# Autodesk Inventor assembly: CubliAssembly2
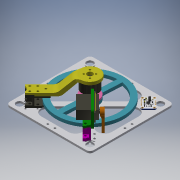
[picture p0: Inventor's stored thumbnail of the model, 180x180]
Saved by Autodesk Inventor 2018 (Build 220112000, 112)
## iProperties
Created: 2019-06-12
Part Number: CubliAssembly2
Document SubType Name: Assembly
Designer: anirudh
Author: anirudh
## Documents named in this file (13)
- C:\Users\anirudh\Documents\MARS Fund\Cubli\CAD Files\CubliAssembly2.iam
- C:\Users\anirudh\Documents\MARS Fund\Cubli\CAD Files\SidePanel.ipt
- C:\Users\anirudh\Documents\MARS Fund\Cubli\CAD Files\MountingBracket.ipt
- C:\Users\anirudh\Documents\MARS Fund\Cubli\CAD Files\MountingArm.ipt
- C:\Users\anirudh\Documents\MARS Fund\Cubli\CAD Files\SnailMotorModel.ipt
- C:\Users\anirudh\Documents\MARS Fund\Cubli\CAD Files\MotorMountingHub.ipt
- C:\Users\anirudh\Documents\MARS Fund\Cubli\CAD Files\AssaultReaper500Servo.ipt
- C:\Users\anirudh\Documents\MARS Fund\Cubli\CAD Files\ServoMount.ipt
- C:\Users\anirudh\Documents\MARS Fund\Cubli\CAD Files\ServoBase.ipt
- C:\Users\anirudh\Documents\MARS Fund\Cubli\CAD Files\Adafruit_BNO055_AP214.ipt
- C:\Users\anirudh\Documents\MARS Fund\Cubli\CAD Files\FlywheelMount.ipt
- C:\Users\anirudh\Documents\MARS Fund\Cubli\CAD Files\AcrylicFlywheels\AcrylicFlywheel3.ipt
- C:\Users\anirudh\Documents\MARS Fund\Cubli\CAD Files\Brake2.ipt
## Components (12 placed, 12 different names)
1. SidePanel:1 — Mate:3, Mate:11, Mate:12, Mate:13, Mate:21, Mate:27, Mate:28, Mate:32, Mate:33, Mate:38, Mate:39
2. MountingBracket:1 — Mate:3, Mate:6, Flush:1, Mate:34, Mate:38, Mate:39
3. MountingArm:1 — Mate:6, Flush:1, Mate:9, Mate:34, Mate:35
4. SnailMotorModel:1 — Mate:7, Mate:8, Mate:9, Mate:35
5. MotorMountingHub:1 — Mate:7, Mate:8
6. AssaultReaper500Servo:1 — Mate:16, Flush:3, Mate:17, Mate:36, Mate:37
7. ServoMount:1 — Mate:14, Flush:2, Mate:15, Mate:16, Flush:3, Mate:17
8. ServoBase:1 — Mate:11, Mate:12, Mate:13, Mate:14, Flush:2, Mate:15
9. Adafruit_BNO055_AP214:1 — Mate:21, Mate:27, Mate:28
10. FlywheelMount:1 — Mate:29, Mate:30, Mate:31
11. AcrylicFlywheel3:1 — Mate:29, Mate:30, Mate:31, Mate:32, Mate:33
12. Brake2:1 — Mate:36, Mate:37
## Relationships (29: Mate 26, Flush 3)
- Mate:3: SidePanel:1 ↔ MountingBracket:1
- Mate:6: MountingBracket:1 ↔ MountingArm:1
- Flush:1: MountingBracket:1 ↔ MountingArm:1
- Mate:7: SnailMotorModel:1 ↔ MotorMountingHub:1
- Mate:8: SnailMotorModel:1 ↔ MotorMountingHub:1
- Mate:9: MountingArm:1 ↔ SnailMotorModel:1
- Mate:11: SidePanel:1 ↔ ServoBase:1
- Mate:12: SidePanel:1 ↔ ServoBase:1
- Mate:13: SidePanel:1 ↔ ServoBase:1
- Mate:14: ServoMount:1 ↔ ServoBase:1
- Flush:2: ServoMount:1 ↔ ServoBase:1
- Mate:15: ServoMount:1 ↔ ServoBase:1
- Mate:16: AssaultReaper500Servo:1 ↔ ServoMount:1
- Flush:3: AssaultReaper500Servo:1 ↔ ServoMount:1
- Mate:17: AssaultReaper500Servo:1 ↔ ServoMount:1
- Mate:21: SidePanel:1 ↔ Adafruit_BNO055_AP214:1
- Mate:27: SidePanel:1 ↔ Adafruit_BNO055_AP214:1
- Mate:28: SidePanel:1 ↔ Adafruit_BNO055_AP214:1
- Mate:29: FlywheelMount:1 ↔ AcrylicFlywheel3:1
- Mate:30: FlywheelMount:1 ↔ AcrylicFlywheel3:1
- Mate:31: FlywheelMount:1 ↔ AcrylicFlywheel3:1
- Mate:32 (6.35 mm): SidePanel:1 ↔ AcrylicFlywheel3:1
- Mate:33: SidePanel:1 ↔ AcrylicFlywheel3:1
- Mate:34: MountingBracket:1 ↔ MountingArm:1
- Mate:35: MountingArm:1 ↔ SnailMotorModel:1
- Mate:36: AssaultReaper500Servo:1 ↔ Brake2:1
- Mate:37: AssaultReaper500Servo:1 ↔ Brake2:1
- Mate:38: SidePanel:1 ↔ MountingBracket:1
- Mate:39: SidePanel:1 ↔ MountingBracket:1
